# Autodesk Inventor assembly: Outer_C_Channel_29
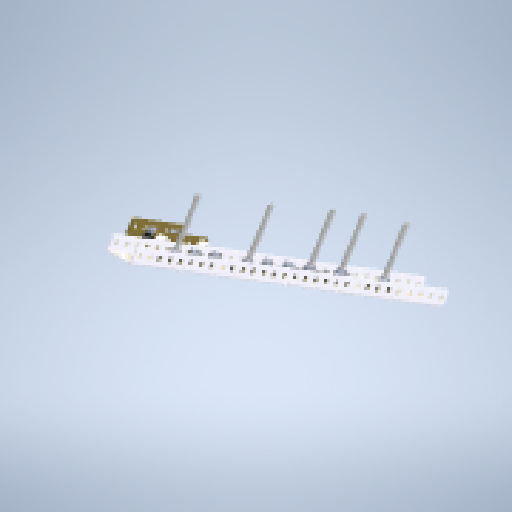
[picture p0: Inventor's stored thumbnail of the model, 512x512]
Saved by Autodesk Inventor 2025.2 (Build 292293000, 293)
## iProperties
Created: 2024-12-08
Part Number: Outer_C_Channel_29
Document SubType Name: Assembly
Designer: Aditya Koduri
Author: Aditya Koduri
## Documents named in this file (12)
- C:\Users\joshi\Desktop\3388K CAD\Outer_C_Channel_30.iam
- C:\Users\joshi\Desktop\3388K CAD\Screw_Joint.iam
- C:\Users\joshi\Desktop\3388K CAD\VEX Main\Motion\Spacers\Spacer Nylon .313 OD\NSpacer .313 OD x .250.ipt
- C:\Users\joshi\Desktop\3388K CAD\VEX Main\Structure\Standoff\Standoff .50.ipt
- C:\Users\joshi\Desktop\3388K CAD\VEX Main\Structure\C Channel\Aluminum 1x2x1\Alu C 1x2x1x5.ipt
- C:\Users\joshi\Desktop\3388K CAD\VEX Main\Motion\Shaft LS\Bearing Flat.ipt
- C:\Users\joshi\Desktop\3388K CAD\VEX Main\Structure\Hardware\Screw Steel - Hex\SScrew Hex Smooth .500.ipt
- C:\Users\joshi\Desktop\3388K CAD\VEX Main\Structure\Hardware\Nut Thin Nylock.ipt
- C:\Users\joshi\Desktop\3388K CAD\VEX Main\Structure\C Channel\Aluminum 1x2x1\Alu C 1x2x1x30.ipt
- C:\Users\mzart\Downloads\VEX-CAD-Inventor-main\VEX-CAD-Inventor-main\Motion\Spacers\Spacer Nylon .313 OD.ipt
- C:\Users\mzart\Downloads\VEX-CAD-Inventor-main\VEX-CAD-Inventor-main\Structure\Standoff.ipt
- C:\Users\mzart\Downloads\VEX-CAD-Inventor-main\VEX-CAD-Inventor-main\Structure\Hardware\Screw Steel - Hex.ipt
## Components (26 placed, 8 different names)
1. Alu C 1x2x1x30:2 — Insert:85, Insert:86, Insert:87, Insert:93, Insert:94, Insert:95, Insert:98, Insert:99, Insert:100, Insert:101, Insert:104, Insert:105, Insert:106, Insert:107, Insert:114
2. Bearing Flat:6 — Insert:96, Insert:97, Insert:110, Insert:111
3. Bearing Flat:7 — Insert:100, Insert:101, Insert:112, Insert:113
4. Screw_Joint:14 [sub-assembly] — Insert:85
5. Screw_Joint:16 [sub-assembly] — Insert:86
6. Screw_Joint:17 [sub-assembly] — Insert:87
7. Alu C 1x2x1x5:2 — Insert:96, Insert:97, Insert:102, Insert:103
8. NSpacer .313 OD x .250:3
9. NSpacer .313 OD x .250:4
10. Standoff .50:3 — Insert:94
11. Standoff .50:4 — Insert:93
12. Bearing Flat:8 — Insert:98, Insert:99, Insert:108, Insert:109
13. Screw_Joint:18 [sub-assembly] — Insert:95
14. Nut Thin Nylock:14 — Insert:113
15. Nut Thin Nylock:15 — Insert:112
16. SScrew Hex Smooth .500:17 — Insert:102
17. SScrew Hex Smooth .500:18 — Insert:107
18. Nut Thin Nylock:16 — Insert:108
19. Nut Thin Nylock:17 — Insert:111
20. SScrew Hex Smooth .500:19 — Insert:104
21. SScrew Hex Smooth .500:20 — Insert:105
22. Nut Thin Nylock:18 — Insert:109
23. Nut Thin Nylock:19 — Insert:110
24. SScrew Hex Smooth .500:21 — Insert:103
25. SScrew Hex Smooth .500:22 — Insert:106
26. Screw_Joint:19 [sub-assembly] — Insert:114
## Relationships (29: Insert 29)
- Insert:85: Alu C 1x2x1x30:2 ↔ Screw_Joint:14
- Insert:86: Alu C 1x2x1x30:2 ↔ Screw_Joint:16
- Insert:87: Alu C 1x2x1x30:2 ↔ Screw_Joint:17
- [Insert]: Alu C 1x2x1x5:2 ↔ NSpacer .313 OD x .250:3
- [Insert]: Alu C 1x2x1x5:2 ↔ NSpacer .313 OD x .250:4
- [Insert]: NSpacer .313 OD x .250:4 ↔ Standoff .50:3
- [Insert]: NSpacer .313 OD x .250:3 ↔ Standoff .50:4
- Insert:93: Alu C 1x2x1x30:2 ↔ Standoff .50:4
- Insert:94: Alu C 1x2x1x30:2 ↔ Standoff .50:3
- Insert:95: Alu C 1x2x1x30:2 ↔ Screw_Joint:18
- Insert:96: Bearing Flat:6 ↔ Alu C 1x2x1x5:2
- Insert:97: Bearing Flat:6 ↔ Alu C 1x2x1x5:2
- Insert:98: Alu C 1x2x1x30:2 ↔ Bearing Flat:8
- Insert:99: Alu C 1x2x1x30:2 ↔ Bearing Flat:8
- Insert:100: Alu C 1x2x1x30:2 ↔ Bearing Flat:7
- Insert:101: Alu C 1x2x1x30:2 ↔ Bearing Flat:7
- Insert:102: Alu C 1x2x1x5:2 ↔ SScrew Hex Smooth .500:17
- Insert:103: Alu C 1x2x1x5:2 ↔ SScrew Hex Smooth .500:21
- Insert:104: Alu C 1x2x1x30:2 ↔ SScrew Hex Smooth .500:19
- Insert:105: Alu C 1x2x1x30:2 ↔ SScrew Hex Smooth .500:20
- Insert:106: Alu C 1x2x1x30:2 ↔ SScrew Hex Smooth .500:22
- Insert:107: Alu C 1x2x1x30:2 ↔ SScrew Hex Smooth .500:18
- Insert:108: Bearing Flat:8 ↔ Nut Thin Nylock:16
- Insert:109: Bearing Flat:8 ↔ Nut Thin Nylock:18
- Insert:110: Bearing Flat:6 ↔ Nut Thin Nylock:19
- Insert:111: Bearing Flat:6 ↔ Nut Thin Nylock:17
- Insert:112: Bearing Flat:7 ↔ Nut Thin Nylock:15
- Insert:113: Bearing Flat:7 ↔ Nut Thin Nylock:14
- Insert:114: Alu C 1x2x1x30:2 ↔ Screw_Joint:19
## Named parameters: d92_d17 = 0 mm, d93_d18 = 0 mm, d94_d19 = 0 mm, d95_d20 = 0 mm
